# Autodesk Inventor assembly: Weapon Assembly
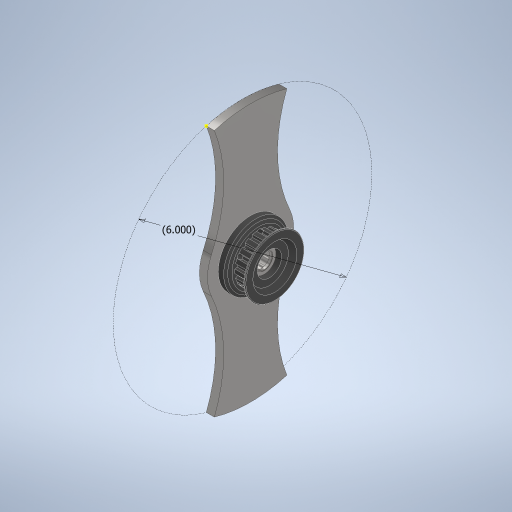
[picture p0: Inventor's stored thumbnail of the model, 512x512]
Saved by Autodesk Inventor 2023.2 (Build 272271000, 271)
## iProperties
Created: 2023-03-06
Part Number: Weapon Assembly
Document SubType Name: Assembly
Designer: Nathan Cai
Author: Nathan Cai
## Documents named in this file (5)
- C:\Users\Nathan Cai\Documents\Inventor\0.3rd Lawette - V3.6\Horizontal Weapon Assembly (Type Spd)\Weapon Assembly.iam
- C:\Users\Nathan Cai\Documents\Inventor\0.3rd Lawette - V3.6\Horizontal Weapon Assembly (Type Spd)\Blade (Bar 2).ipt
- C:\Users\Nathan Cai\Documents\Inventor\0.3rd Lawette - V3.6\Horizontal Weapon Assembly (Type Spd)\Spacer 3-8x .125.ipt
- C:\Users\Nathan Cai\Documents\Inventor\0.3rd Lawette - V3.6\Horizontal Weapon Assembly (Type Spd)\5905K132_Needle-Roller Bearing.ipt
- C:\Users\Nathan Cai\Documents\Inventor\0.3rd Lawette - V3.6\Horizontal Weapon Assembly (Type Spd)\XL Pulley 18T .25in Wd.ipt
## Components (4 placed, 4 different names)
1. Blade (Bar 2):1 — Mate:1, Mate:2, Mate:3, Mate:4, Mate:5, Mate:6
2. Spacer 3-8x .125:1 — Mate:1, Mate:2, Mate:3, Flush:1
3. 5905K132_Needle-Roller Bearing:1 — Mate:4, Flush:1, Mate:7
4. XL Pulley 18T .25in Wd:1 — Mate:5, Mate:6, Mate:7
## Relationships (8: Mate 7, Flush 1)
- Mate:1: Blade (Bar 2):1 ↔ Spacer 3-8x .125:1
- Mate:2: Blade (Bar 2):1 ↔ Spacer 3-8x .125:1
- Mate:3: Blade (Bar 2):1 ↔ Spacer 3-8x .125:1
- Mate:4: Blade (Bar 2):1 ↔ 5905K132_Needle-Roller Bearing:1
- Flush:1: Spacer 3-8x .125:1 ↔ 5905K132_Needle-Roller Bearing:1
- Mate:5: Blade (Bar 2):1 ↔ XL Pulley 18T .25in Wd:1
- Mate:6: Blade (Bar 2):1 ↔ XL Pulley 18T .25in Wd:1
- Mate:7: 5905K132_Needle-Roller Bearing:1 ↔ XL Pulley 18T .25in Wd:1
